# Autodesk Inventor assembly: Assembly1
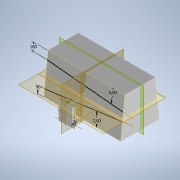
[picture p0: Inventor's stored thumbnail of the model, 180x180]
Saved by Autodesk Inventor 2021 (Build 250183000, 183)
## iProperties
Created: 2021-05-04
Part Number: Assembly1
Document SubType Name: Assembly
Designer: andre
Author: andre
## Documents named in this file (5)
- C:\Users\andre\Desktop\DYNAMIS 2021\Riunioni - Corsi\Corsi Academy\Multibody-Suspension\CAD files\Inventor\Assembly1.iam
- C:\Users\andre\Desktop\DYNAMIS 2021\Riunioni - Corsi\Corsi Academy\Multibody-Suspension\CAD files\Inventor\Telaio.ipt
- C:\Users\andre\Desktop\DYNAMIS 2021\Riunioni - Corsi\Corsi Academy\Multibody-Suspension\CAD files\Inventor\Braccetto.ipt
- C:\Users\andre\Desktop\DYNAMIS 2021\Riunioni - Corsi\Corsi Academy\Multibody-Suspension\CAD files\Inventor\hub.ipt
- C:\Users\andre\Desktop\DYNAMIS 2021\Riunioni - Corsi\Corsi Academy\Multibody-Suspension\CAD files\Inventor\tie.ipt
## Components (5 placed, 4 different names)
1. Telaio:1 — Flush:1, Flush:2, Flush:3, Mate:1, Mate:3
2. Braccetto:1 — Mate:1, Mate:10, Mate:13
3. Braccetto:2 — Mate:3, Mate:12, Mate:14, Mate:16
4. hub:1 — Mate:10, Mate:14, Mate:17
5. tie:1 — Mate:16, Mate:17
## Relationships (11: Mate 8, Flush 3)
- Flush:1: Telaio:1
- Flush:2: Telaio:1
- Flush:3: Telaio:1
- Mate:1: Telaio:1 ↔ Braccetto:1
- Mate:3: Telaio:1 ↔ Braccetto:2
- Mate:10: Braccetto:1 ↔ hub:1
- Mate:12: Braccetto:2
- Mate:13: Braccetto:1
- Mate:14: Braccetto:2 ↔ hub:1
- Mate:16: Braccetto:2 ↔ tie:1
- Mate:17: hub:1 ↔ tie:1
